# Autodesk Inventor assembly: Jig_assembly
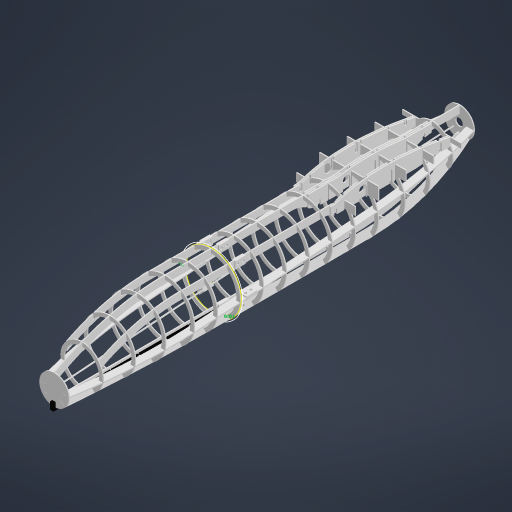
[picture p0: Inventor's stored thumbnail of the model, 512x512]
Saved by Autodesk Inventor 2023 (Build 270158000, 158)
## iProperties
Created: 2023-05-07
Part Number: Jig_assembly
Document SubType Name: Assembly
Designer: szykr
Author: szykr
## Documents named in this file (4)
- D:\Folder Instalacyjny\GitHub Pliki\Solaris\new model\Jig\Jig_assembly.iam
- D:\Folder Instalacyjny\GitHub Pliki\Solaris\new model\nowy kadłub.ipt
- D:\Folder Instalacyjny\GitHub Pliki\Solaris\new model\Jig\Jig_1.ipt
- D:\Folder Instalacyjny\GitHub Pliki\Solaris\new model\Jig\Front_aligner.ipt
## Components (3 placed, 3 different names)
1. nowy kadłub:1 — Flush:2
2. Jig_1:1 — Flush:1
3. Front_aligner:1 — Flush:2
## Relationships (2: Flush 2)
- Flush:1: Jig_1:1
- Flush:2: nowy kadłub:1 ↔ Front_aligner:1
